# Autodesk Inventor assembly: Gears
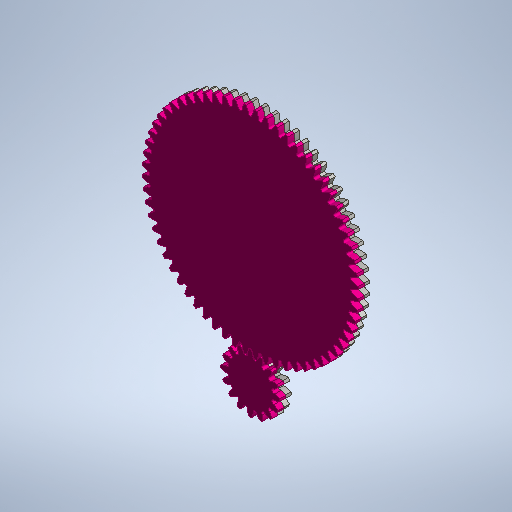
[picture p0: Inventor's stored thumbnail of the model, 512x512]
Saved by Autodesk Inventor 2025 (Build 290162010, 162A)
## iProperties
Part Number: Gears
Document SubType Name: Assembly
Designer: pokla
Author: pokla
## Documents named in this file (4)
- C:\Users\pokla\Documents\Inventor\ДФО\ДМФ\DMF-Disk-Micro-Filter\Новые шестерни 27.08.2025\Gears.iam
- C:\Users\pokla\Documents\Inventor\ДФО\ДМФ\DMF-Disk-Micro-Filter\Новые шестерни 27.08.2025\Gears\Design Accelerator\Spur Gears1.iam
- C:\Users\pokla\Documents\Inventor\ДФО\ДМФ\DMF-Disk-Micro-Filter\Новые шестерни 27.08.2025\big gear.ipt
- C:\Users\pokla\Documents\Inventor\ДФО\ДМФ\DMF-Disk-Micro-Filter\Новые шестерни 27.08.2025\small gear.ipt
## Components (3 placed, 3 different names)
1. Spur Gears:1 [sub-assembly] — Rotational:1, Rotational:2
2. big gear:1 — Rotational:1
3. small gear:1 — Rotational:2
## Relationships (2: RevoluteJoint 2)
- Rotational:1 [RevoluteJoint]: Spur Gears:1 ↔ big gear:1
- Rotational:2 [RevoluteJoint]: Spur Gears:1 ↔ small gear:1
